# Autodesk Inventor assembly: TestSetup
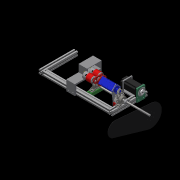
[picture p0: Inventor's stored thumbnail of the model, 180x180]
Saved by Autodesk Inventor 2018 (Build 220112000, 112)
## iProperties
Created: 2021-12-07
Part Number: TestSetup
Document SubType Name: Assembly
Designer: kumpu
Author: kumpu
## Documents named in this file (29)
- C:\Users\kumpu\Documents\SBU\CAD\SBRT\Robocup Rescue\Drive\TestSetup1\TestSetup1.iam
- C:\Users\kumpu\Documents\SBU\CAD\SBRT\Robocup Rescue\Drive\TestSetup1\am-0237 60T 25 Chain Bearing Bore Sprocket.ipt
- C:\Users\kumpu\Documents\SBU\CAD\SBRT\Robocup Rescue\Drive\TestSetup1\am-2201 Gear 48 Tooth, 20 dp, 500 Key Bore.ipt
- C:\Users\kumpu\Documents\SBU\CAD\SBRT\Robocup Rescue\Drive\TestSetup1\am-4212 18T 20DP 500hex 375 FW.ipt
- C:\Users\kumpu\Documents\SBU\CAD\SBRT\Robocup Rescue\Drive\TestSetup1\am-4465 1-2 in ID 1 1-8 in OD Sealed Flanged Bearing FR82RS.ipt
- C:\Users\kumpu\Documents\SBU\CAD\SBRT\Robocup Rescue\Drive\TestSetup1\5913K61_Low-Profile Mounted Sealed Steel Ball Bearing.ipt
- C:\Users\kumpu\Documents\SBU\CAD\SBRT\Robocup Rescue\Drive\TestSetup1\am-3620 - S25-24HA-500K.ipt
- C:\Users\kumpu\Documents\SBU\CAD\SBRT\Robocup Rescue\Drive\TestSetup1\am-3692 DeCIMate Output Plate.ipt
- C:\Users\kumpu\Documents\SBU\CAD\SBRT\Robocup Rescue\Drive\TestSetup1\am-3693 DeCIMate Motor Plate.ipt
- C:\Users\kumpu\Documents\SBU\CAD\SBRT\Robocup Rescue\Drive\TestSetup1\am-3650 775 Motor Vent Plate.ipt
- C:\Users\kumpu\Documents\SBU\CAD\SBRT\Robocup Rescue\Drive\TestSetup1\am-3775a AndyMark RedLine Motor.ipt
- C:\Users\kumpu\Documents\SBU\CAD\SBRT\Robocup Rescue\Drive\TestSetup1\am-0028 00.375'' id Flanged, Shielded Ball Bearing (FR6ZZ).ipt
- C:\Users\kumpu\Documents\SBU\CAD\SBRT\Robocup Rescue\Drive\TestSetup1\am-3695 DeCIMate Output Shaft.ipt
- C:\Users\kumpu\Documents\SBU\CAD\SBRT\Robocup Rescue\Drive\TestSetup1\6627T55_Position-Control DC Motor.ipt
- C:\Users\kumpu\Documents\SBU\CAD\SBRT\Robocup Rescue\Drive\TestSetup1\base2.ipt
- C:\Users\kumpu\Documents\SBU\CAD\SBRT\Robocup Rescue\Drive\TestSetup1\base5.ipt
- C:\Users\kumpu\Documents\SBU\CAD\SBRT\Robocup Rescue\Drive\TestSetup1\RCR_drive_test_flipper.ipt
- C:\Users\kumpu\Documents\SBU\CAD\SBRT\Robocup Rescue\Drive\TestSetup1\StepperAdapter.ipt
- C:\Users\kumpu\Documents\SBU\CAD\SBRT\Robocup Rescue\Drive\TestSetup1\M3.ipt
- C:\Users\kumpu\Documents\SBU\CAD\SBRT\Robocup Rescue\Drive\TestSetup1\3 Stage HD - CIM Sport_Shrinkwrap_1.ipt
- C:\Users\kumpu\Documents\SBU\CAD\SBRT\Robocup Rescue\Drive\TestSetup1\S3_ph.ipt
- C:\Users\kumpu\Documents\SBU\CAD\SBRT\Robocup Rescue\Drive\TestSetup1\S4.ipt
- C:\Users\kumpu\Documents\SBU\CAD\SBRT\Robocup Rescue\Drive\TestSetup1\M1 mk1.ipt
- C:\Users\kumpu\Documents\SBU\CAD\SBRT\Robocup Rescue\Drive\TestSetup1\spacer_S2.ipt
- C:\Users\kumpu\Documents\SBU\CAD\SBRT\Robocup Rescue\Drive\TestSetup1\M2_spacer.ipt
- C:\Users\kumpu\Documents\SBU\CAD\SBRT\Robocup Rescue\Drive\TestSetup1\M2_plate.ipt
- C:\Users\kumpu\Documents\SBU\CAD\SBRT\Robocup Rescue\Drive\TestSetup1\Axle.ipt
- C:\Users\kumpu\Documents\SBU\CAD\SBRT\Robocup Rescue\Drive\TestSetup1\B1_RCR_v1.ipt
- C:\Users\kumpu\Documents\SBU\CAD\SBRT\Robocup Rescue\Drive\TestSetup1\B2_RCR_v1.ipt
## Components (34 placed, 28 different names)
1. 3 Stage HD - CIM Sport_Shrinkwrap_1:1 — Flush:1, Mate:1, Angle:1, Insert:1, Angle:2, Mate:2, Mate:13, Angle:5, Mate:14
2. am-0237 60T 25 Chain Bearing Bore Sprocket:1 — Angle:4, Insert:3, Flush:8, Mate:23, Insert:21
3. am-2201 Gear 48 Tooth, 20 dp, 500 Key Bore:1 — Flush:2, Mate:2, Mate:3, Mate:8, Mate:19, Mate:21, Mate:26, Mate:34
4. am-4212 18T 20DP 500hex 375 FW:1 — Insert:1, Angle:2, Flush:2
5. am-4465 1-2 in ID 1 1-8 in OD Sealed Flanged Bearing FR82RS:1 — Insert:3, Mate:4, Mate:22, Insert:24
6. 5913K61_Low-Profile Mounted Sealed Steel Ball Bearing:1 — Mate:4, Flush:3, Mate:8, Angle:8, Mate:26, Mate:33, Insert:26
7. 5913K61_Low-Profile Mounted Sealed Steel Ball Bearing:2 — Flush:3, Flush:10, Mate:17, Mate:19, Mate:20, Mate:21, Mate:25
8. am-3620 - S25-24HA-500K:1 — Flush:8, Mate:7, Angle:7, Insert:18
9. am-3692 DeCIMate Output Plate:1 — Insert:5, Insert:6, Mate:13, Mate:14
10. am-3693 DeCIMate Motor Plate:1 — Insert:5, Insert:6, Insert:7, Insert:8, Insert:9, Insert:10, Angle:5, Insert:15, Angle:8
11. am-3650 775 Motor Vent Plate:1 — Insert:8, Insert:9, Insert:11, Insert:12
12. am-3775a AndyMark RedLine Motor:1 — Insert:13, Insert:14
13. am-3650 775 Motor Vent Plate:2 — Insert:7, Insert:10, Insert:13, Insert:14
14. am-3775a AndyMark RedLine Motor:2 — Insert:11, Insert:12
15. am-0028 00.375'' id Flanged, Shielded Ball Bearing (FR6ZZ):1 — Insert:15, Insert:16
16. am-3695 DeCIMate Output Shaft:1 — Insert:16
17. 6627T55_Position-Control DC Motor:1 — Mate:7, Angle:6, Flush:10, Flush:11, Angle:7, Flush:17, Mate:39, Mate:40
18. base2:1 — Mate:15, Flush:13, Flush:14, Mate:17, Flush:11, Mate:20, Mate:27, Angle:9, Mate:28, Flush:19, Mate:35, Mate:37
19. base2:2 — Mate:16, Flush:12, Flush:15
20. base5:1 — Mate:15, Mate:16, Flush:12, Flush:13, Flush:14, Flush:15, Mate:25, Mate:32, Flush:18, Mate:38, Flush:20
21. RCR_drive_test_flipper:1 — Mate:22, Mate:23, Insert:17, Insert:19, Insert:20, Mate:30, Mate:31, Insert:25, Mate:36
22. am-4465 1-2 in ID 1 1-8 in OD Sealed Flanged Bearing FR82RS:2 — Insert:17
23. StepperAdapter:1 — Insert:18, Flush:17, Mate:29
24. M3:1 — Mate:27, Angle:9, Mate:28, Mate:29
25. S3_ph:1 — Insert:20, Insert:21, Mate:31
26. S4:1 — Insert:19, Mate:30
27. M1 mk1:1 — Mate:32, Flush:18, Mate:33
28. RCR_drive_test_flipper:2 — Insert:25, Mate:36
29. spacer_S2:1 — Insert:24
30. M2_spacer:1 — Insert:22, Insert:23, Mate:34, Flush:19, Mate:35
31. M2_plate:1 — Insert:22, Insert:23
32. Axle:1 — Insert:26
33. B1_RCR_v1:1 — Mate:38, Flush:20
34. B2_RCR_v1:1 — Mate:37, Mate:39, Mate:40
## Relationships (78: Mate 32, Insert 24, Flush 14, Angle 8)
- Flush:1: 3 Stage HD - CIM Sport_Shrinkwrap_1:1
- Mate:1: 3 Stage HD - CIM Sport_Shrinkwrap_1:1
- Angle:1 (-45 deg): 3 Stage HD - CIM Sport_Shrinkwrap_1:1
- Insert:1: 3 Stage HD - CIM Sport_Shrinkwrap_1:1 ↔ am-4212 18T 20DP 500hex 375 FW:1
- Angle:2 (0 deg): 3 Stage HD - CIM Sport_Shrinkwrap_1:1 ↔ am-4212 18T 20DP 500hex 375 FW:1
- Flush:2: am-2201 Gear 48 Tooth, 20 dp, 500 Key Bore:1 ↔ am-4212 18T 20DP 500hex 375 FW:1
- Mate:2 (41.91 mm): 3 Stage HD - CIM Sport_Shrinkwrap_1:1 ↔ am-2201 Gear 48 Tooth, 20 dp, 500 Key Bore:1
- Mate:3: am-2201 Gear 48 Tooth, 20 dp, 500 Key Bore:1
- Angle:4 (0 deg): am-0237 60T 25 Chain Bearing Bore Sprocket:1
- Insert:3: am-0237 60T 25 Chain Bearing Bore Sprocket:1 ↔ am-4465 1-2 in ID 1 1-8 in OD Sealed Flanged Bearing FR82RS:1
- Mate:4: am-4465 1-2 in ID 1 1-8 in OD Sealed Flanged Bearing FR82RS:1 ↔ 5913K61_Low-Profile Mounted Sealed Steel Ball Bearing:1
- Flush:17: 6627T55_Position-Control DC Motor:1 ↔ StepperAdapter:1
- Flush:3: 5913K61_Low-Profile Mounted Sealed Steel Ball Bearing:1 ↔ 5913K61_Low-Profile Mounted Sealed Steel Ball Bearing:2
- Flush:8: am-0237 60T 25 Chain Bearing Bore Sprocket:1 ↔ am-3620 - S25-24HA-500K:1
- Insert:5 (19.05 mm): am-3692 DeCIMate Output Plate:1 ↔ am-3693 DeCIMate Motor Plate:1
- Insert:6 (19.05 mm): am-3692 DeCIMate Output Plate:1 ↔ am-3693 DeCIMate Motor Plate:1
- Insert:7: am-3693 DeCIMate Motor Plate:1 ↔ am-3650 775 Motor Vent Plate:2
- Insert:8: am-3693 DeCIMate Motor Plate:1 ↔ am-3650 775 Motor Vent Plate:1
- Insert:9: am-3693 DeCIMate Motor Plate:1 ↔ am-3650 775 Motor Vent Plate:1
- Insert:10: am-3693 DeCIMate Motor Plate:1 ↔ am-3650 775 Motor Vent Plate:2
- Insert:11: am-3650 775 Motor Vent Plate:1 ↔ am-3775a AndyMark RedLine Motor:2
- Insert:12: am-3650 775 Motor Vent Plate:1 ↔ am-3775a AndyMark RedLine Motor:2
- Insert:13: am-3775a AndyMark RedLine Motor:1 ↔ am-3650 775 Motor Vent Plate:2
- Insert:14: am-3775a AndyMark RedLine Motor:1 ↔ am-3650 775 Motor Vent Plate:2
- Mate:13: 3 Stage HD - CIM Sport_Shrinkwrap_1:1 ↔ am-3692 DeCIMate Output Plate:1
- Angle:5 (45 deg): 3 Stage HD - CIM Sport_Shrinkwrap_1:1 ↔ am-3693 DeCIMate Motor Plate:1
- Insert:15: am-3693 DeCIMate Motor Plate:1 ↔ am-0028 00.375'' id Flanged, Shielded Ball Bearing (FR6ZZ):1
- Insert:16: am-0028 00.375'' id Flanged, Shielded Ball Bearing (FR6ZZ):1 ↔ am-3695 DeCIMate Output Shaft:1
- Mate:7: am-3620 - S25-24HA-500K:1 ↔ 6627T55_Position-Control DC Motor:1
- Angle:6 (0 deg): 6627T55_Position-Control DC Motor:1
- Flush:10: 5913K61_Low-Profile Mounted Sealed Steel Ball Bearing:2 ↔ 6627T55_Position-Control DC Motor:1
- Mate:8: am-2201 Gear 48 Tooth, 20 dp, 500 Key Bore:1 ↔ 5913K61_Low-Profile Mounted Sealed Steel Ball Bearing:1
- Flush:11: 6627T55_Position-Control DC Motor:1 ↔ base2:1
- Mate:14: 3 Stage HD - CIM Sport_Shrinkwrap_1:1 ↔ am-3692 DeCIMate Output Plate:1
- Mate:15: base2:1 ↔ base5:1
- Mate:16: base2:2 ↔ base5:1
- Flush:12: base2:2 ↔ base5:1
- Flush:13: base2:1 ↔ base5:1
- Flush:14: base2:1 ↔ base5:1
- Flush:15: base2:2 ↔ base5:1
- Mate:17: 5913K61_Low-Profile Mounted Sealed Steel Ball Bearing:2 ↔ base2:1
- Angle:7 (0 deg): am-3620 - S25-24HA-500K:1 ↔ 6627T55_Position-Control DC Motor:1
- Mate:19: am-2201 Gear 48 Tooth, 20 dp, 500 Key Bore:1 ↔ 5913K61_Low-Profile Mounted Sealed Steel Ball Bearing:2
- Mate:20 (-15 mm): 5913K61_Low-Profile Mounted Sealed Steel Ball Bearing:2 ↔ base2:1
- Mate:21: am-2201 Gear 48 Tooth, 20 dp, 500 Key Bore:1 ↔ 5913K61_Low-Profile Mounted Sealed Steel Ball Bearing:2
- Angle:8 (0 deg): 5913K61_Low-Profile Mounted Sealed Steel Ball Bearing:1 ↔ am-3693 DeCIMate Motor Plate:1
- Mate:22: am-4465 1-2 in ID 1 1-8 in OD Sealed Flanged Bearing FR82RS:1 ↔ RCR_drive_test_flipper:1
- Mate:23: am-0237 60T 25 Chain Bearing Bore Sprocket:1 ↔ RCR_drive_test_flipper:1
- Mate:25 (12.7 mm): 5913K61_Low-Profile Mounted Sealed Steel Ball Bearing:2 ↔ base5:1
- Insert:17 (1.27 mm): RCR_drive_test_flipper:1 ↔ am-4465 1-2 in ID 1 1-8 in OD Sealed Flanged Bearing FR82RS:2
- Mate:26 (139.7 mm): am-2201 Gear 48 Tooth, 20 dp, 500 Key Bore:1 ↔ 5913K61_Low-Profile Mounted Sealed Steel Ball Bearing:1
- Insert:18: am-3620 - S25-24HA-500K:1 ↔ StepperAdapter:1
- Mate:27 (-15 mm): base2:1 ↔ M3:1
- Angle:9 (0 deg): base2:1 ↔ M3:1
- Mate:28: base2:1 ↔ M3:1
- Mate:29: StepperAdapter:1 ↔ M3:1
- Insert:19: RCR_drive_test_flipper:1 ↔ S4:1
- Insert:20: RCR_drive_test_flipper:1 ↔ S3_ph:1
- Insert:21: am-0237 60T 25 Chain Bearing Bore Sprocket:1 ↔ S3_ph:1
- Mate:30 (0.254 mm): RCR_drive_test_flipper:1 ↔ S4:1
- Mate:31 (0.254 mm): RCR_drive_test_flipper:1 ↔ S3_ph:1
- Mate:32: base5:1 ↔ M1 mk1:1
- Flush:18: base5:1 ↔ M1 mk1:1
- Mate:33: 5913K61_Low-Profile Mounted Sealed Steel Ball Bearing:1 ↔ M1 mk1:1
- Insert:22: M2_spacer:1 ↔ M2_plate:1
- Insert:23: M2_spacer:1 ↔ M2_plate:1
- Mate:34: am-2201 Gear 48 Tooth, 20 dp, 500 Key Bore:1 ↔ M2_spacer:1
- Flush:19: base2:1 ↔ M2_spacer:1
- Mate:35: base2:1 ↔ M2_spacer:1
- Insert:24: am-4465 1-2 in ID 1 1-8 in OD Sealed Flanged Bearing FR82RS:1 ↔ spacer_S2:1
- Insert:25 (88.9 mm): RCR_drive_test_flipper:1 ↔ RCR_drive_test_flipper:2
- Mate:36: RCR_drive_test_flipper:1 ↔ RCR_drive_test_flipper:2
- Insert:26 (-25.4 mm): 5913K61_Low-Profile Mounted Sealed Steel Ball Bearing:1 ↔ Axle:1
- Mate:37: base2:1 ↔ B2_RCR_v1:1
- Mate:38: base5:1 ↔ B1_RCR_v1:1
- Flush:20: base5:1 ↔ B1_RCR_v1:1
- Mate:39: 6627T55_Position-Control DC Motor:1 ↔ B2_RCR_v1:1
- Mate:40: 6627T55_Position-Control DC Motor:1 ↔ B2_RCR_v1:1
